# Autodesk Inventor assembly: TT_Intake
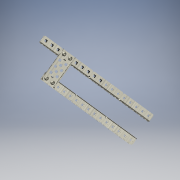
[picture p0: Inventor's stored thumbnail of the model, 180x180]
Saved by Autodesk Inventor 2019 (Build 230136000, 136)
## iProperties
Created: 2020-02-10
Part Number: TT_Intake
Document SubType Name: Assembly
Designer: clove
Author: clove
## Documents named in this file (7)
- C:\Users\clove\Downloads\TT_Intake.iam
- C:\Users\clove\Downloads\SID Library-20181221T040531Z-001\2018 BNS-VRC-SID Library\Structure\C-Channels\C-Channel 1x2x1\Aluminum C-Channel 1x2x1x18.ipt
- C:\Users\clove\Downloads\SID Library-20181221T040531Z-001\2018 BNS-VRC-SID Library\Structure\C-Channels\C-Channel 1x2x1\Aluminum C-Channel 1x2x1x15.ipt
- C:\Users\clove\Downloads\SID Library-20181221T040531Z-001\2018 BNS-VRC-SID Library\Structure\C-Channels\C-Channel 1x2x1\Aluminum C-Channel 1x2x1x5.ipt
- C:\Users\clove\Downloads\SID Library-20181221T040531Z-001\2018 BNS-VRC-SID Library\Structure\Screws _ Nuts\Screw 8-32 x 0.375_.ipt
- C:\Users\clove\Downloads\SID Library-20181221T040531Z-001\2018 BNS-VRC-SID Library\Structure\Screws _ Nuts\8-32 Nylon-Insert Thin Hex Locknut.iam
- C:\Users\clove\Downloads\SID Library-20181221T040531Z-001\2018 BNS-VRC-SID Library\Motion\Bearing Flat.ipt
## Components (14 placed, 6 different names)
1. Aluminum C-Channel 1x2x1x18:1 — Insert:3, Insert:4, Insert:9, Insert:10, Insert:13, Insert:14, Insert:15, Insert:16, Insert:17, Insert:18, Insert:19
2. Aluminum C-Channel 1x2x1x15:1 — Insert:1, Insert:2, Insert:11, Insert:12
3. Aluminum C-Channel 1x2x1x5:1 — Insert:1, Insert:2, Insert:3, Insert:4, Insert:5, Insert:6, Insert:7, Insert:8
4. Screw 8-32 x 0.375_:1 — Insert:5
5. Screw 8-32 x 0.375_:2 — Insert:6
6. Screw 8-32 x 0.375_:3 — Insert:7
7. Screw 8-32 x 0.375_:4 — Insert:8
8. 8-32 Nylon-Insert Thin Hex Locknut:1 [sub-assembly] — Insert:9
9. 8-32 Nylon-Insert Thin Hex Locknut:2 [sub-assembly] — Insert:10
10. 8-32 Nylon-Insert Thin Hex Locknut:3 [sub-assembly] — Insert:11
11. 8-32 Nylon-Insert Thin Hex Locknut:4 [sub-assembly] — Insert:12
12. Bearing Flat:1 — Insert:13, Insert:14
13. Bearing Flat:2 — Insert:15, Insert:16
14. Bearing Flat:3 — Insert:17, Insert:18, Insert:19
## Relationships (19: Insert 19)
- Insert:1: Aluminum C-Channel 1x2x1x15:1 ↔ Aluminum C-Channel 1x2x1x5:1
- Insert:2: Aluminum C-Channel 1x2x1x15:1 ↔ Aluminum C-Channel 1x2x1x5:1
- Insert:3: Aluminum C-Channel 1x2x1x18:1 ↔ Aluminum C-Channel 1x2x1x5:1
- Insert:4: Aluminum C-Channel 1x2x1x18:1 ↔ Aluminum C-Channel 1x2x1x5:1
- Insert:5: Aluminum C-Channel 1x2x1x5:1 ↔ Screw 8-32 x 0.375_:1
- Insert:6: Aluminum C-Channel 1x2x1x5:1 ↔ Screw 8-32 x 0.375_:2
- Insert:7: Aluminum C-Channel 1x2x1x5:1 ↔ Screw 8-32 x 0.375_:3
- Insert:8: Aluminum C-Channel 1x2x1x5:1 ↔ Screw 8-32 x 0.375_:4
- Insert:9: Aluminum C-Channel 1x2x1x18:1 ↔ 8-32 Nylon-Insert Thin Hex Locknut:1
- Insert:10: Aluminum C-Channel 1x2x1x18:1 ↔ 8-32 Nylon-Insert Thin Hex Locknut:2
- Insert:11: Aluminum C-Channel 1x2x1x15:1 ↔ 8-32 Nylon-Insert Thin Hex Locknut:3
- Insert:12: Aluminum C-Channel 1x2x1x15:1 ↔ 8-32 Nylon-Insert Thin Hex Locknut:4
- Insert:13: Aluminum C-Channel 1x2x1x18:1 ↔ Bearing Flat:1
- Insert:14: Aluminum C-Channel 1x2x1x18:1 ↔ Bearing Flat:1
- Insert:15: Aluminum C-Channel 1x2x1x18:1 ↔ Bearing Flat:2
- Insert:16: Aluminum C-Channel 1x2x1x18:1 ↔ Bearing Flat:2
- Insert:17: Aluminum C-Channel 1x2x1x18:1 ↔ Bearing Flat:3
- Insert:18: Aluminum C-Channel 1x2x1x18:1 ↔ Bearing Flat:3
- Insert:19: Aluminum C-Channel 1x2x1x18:1 ↔ Bearing Flat:3
